# Autodesk Inventor assembly: Assembly2
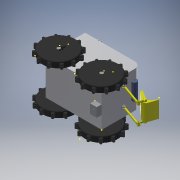
[picture p0: Inventor's stored thumbnail of the model, 180x180]
Saved by Autodesk Inventor 2018 (Build 220112000, 112)
## iProperties
Created: 2018-01-20
Part Number: Assembly2
Document SubType Name: Assembly
Designer: abdul
Author: abdul
## Documents named in this file (13)
- C:\Users\abdul\Desktop\Designathon new\Assembly2.iam
- C:\Users\abdul\Desktop\Designathon new\Design.ipt
- C:\Users\abdul\Desktop\Designathon new\motor.ipt
- C:\Users\abdul\Desktop\Designathon new\battery.ipt
- C:\Users\abdul\Desktop\Designathon new\spiked-wheel.ipt
- C:\Users\abdul\Desktop\Designathon new\rod.ipt
- C:\Users\abdul\Desktop\Designathon new\conveyer belt.ipt
- C:\Users\abdul\Desktop\Designathon new\Sensor.ipt
- C:\Users\abdul\Desktop\Designathon new\robotarm.ipt
- C:\Users\abdul\Desktop\Designathon new\stick.ipt
- C:\Users\abdul\Desktop\Designathon new\hoe me.ipt
- C:\Users\abdul\Desktop\Designathon new\extenstion.ipt
- C:\Users\abdul\Desktop\Designathon new\long extention.ipt
## Components (22 placed, 12 different names)
1. Design:1 — Mate:12, Mate:13, Mate:14, Mate:15, Mate:18, Mate:22, Mate:23, Mate:24, Mate:25, Flush:5, Mate:26, Flush:6, Mate:27, Mate:28, Flush:7, Mate:29, Mate:30, Angle:1, Mate:42, Mate:45, Mate:46, Mate:47, Mate:48, Mate:49
2. motor:1 — Mate:22
3. battery:1 — Mate:12, Mate:13
4. spiked-wheel:1 — Mate:17, Flush:4
5. spiked-wheel:2 — Flush:2, Mate:19
6. spiked-wheel:3 — Mate:16, Flush:3
7. spiked-wheel:4 — Mate:20, Mate:21, Angle:2
8. rod:1 — Mate:14, Mate:16, Flush:3, Mate:17, Flush:4
9. rod:2 — Flush:2, Mate:15, Mate:18, Mate:19, Mate:20, Mate:21
10. conveyer belt:1 — Mate:23, Mate:24, Mate:27
11. Sensor:1 — Mate:25, Flush:5
12. Sensor:2 — Mate:26, Flush:6
13. Sensor:3 — Mate:28, Flush:7
14. robotarm:1 — Mate:29, Mate:30
15. stick:1 — Angle:1, Mate:40, Mate:42, Mate:43, Mate:45, Mate:46
16. stick:2
17. stick:3 — Angle:2, Mate:41, Mate:44, Mate:47, Mate:48, Mate:49
18. hoe me:1 — Mate:33, Mate:36, Mate:37, Mate:38, Mate:39, Flush:8
19. extenstion:1 — Mate:33, Mate:39, Flush:8
20. extenstion:2 — Mate:36, Mate:37, Mate:38, Mate:50, Flush:9, Flush:10
21. long extention:1 — Mate:41, Mate:44, Angle:3
22. long extention:2 — Mate:40, Mate:43, Mate:50, Flush:9, Flush:10, Angle:3
## Relationships (47: Mate 35, Flush 9, Angle 3)
- Mate:12: Design:1 ↔ battery:1
- Mate:13: Design:1 ↔ battery:1
- Flush:2: spiked-wheel:2 ↔ rod:2
- Mate:14: Design:1 ↔ rod:1
- Mate:15: Design:1 ↔ rod:2
- Mate:16: spiked-wheel:3 ↔ rod:1
- Flush:3: spiked-wheel:3 ↔ rod:1
- Mate:17: spiked-wheel:1 ↔ rod:1
- Flush:4: spiked-wheel:1 ↔ rod:1
- Mate:18: Design:1 ↔ rod:2
- Mate:19: spiked-wheel:2 ↔ rod:2
- Mate:20: spiked-wheel:4 ↔ rod:2
- Mate:21: spiked-wheel:4 ↔ rod:2
- Mate:22: Design:1 ↔ motor:1
- Mate:23 (200 mm): Design:1 ↔ conveyer belt:1
- Mate:24 (200 mm): Design:1 ↔ conveyer belt:1
- Mate:25: Design:1 ↔ Sensor:1
- Flush:5: Design:1 ↔ Sensor:1
- Mate:26: Design:1 ↔ Sensor:2
- Flush:6: Design:1 ↔ Sensor:2
- Mate:27 (400 mm): Design:1 ↔ conveyer belt:1
- Mate:28: Design:1 ↔ Sensor:3
- Flush:7: Design:1 ↔ Sensor:3
- Mate:29: Design:1 ↔ robotarm:1
- Mate:30: Design:1 ↔ robotarm:1
- Angle:1 (0 deg): Design:1 ↔ stick:1
- Angle:2 (0 deg): spiked-wheel:4 ↔ stick:3
- Mate:33: hoe me:1 ↔ extenstion:1
- Mate:36: hoe me:1 ↔ extenstion:2
- Mate:37: hoe me:1 ↔ extenstion:2
- Mate:38: hoe me:1 ↔ extenstion:2
- Mate:39: hoe me:1 ↔ extenstion:1
- Flush:8: hoe me:1 ↔ extenstion:1
- Mate:40: stick:1 ↔ long extention:2
- Mate:41: stick:3 ↔ long extention:1
- Mate:42: Design:1 ↔ stick:1
- Mate:43: stick:1 ↔ long extention:2
- Mate:44: stick:3 ↔ long extention:1
- Mate:45: Design:1 ↔ stick:1
- Mate:46: Design:1 ↔ stick:1
- Mate:47: Design:1 ↔ stick:3
- Mate:48: Design:1 ↔ stick:3
- Mate:49: Design:1 ↔ stick:3
- Mate:50: extenstion:2 ↔ long extention:2
- Flush:9: extenstion:2 ↔ long extention:2
- Flush:10: extenstion:2 ↔ long extention:2
- Angle:3 (0 deg): long extention:1 ↔ long extention:2
